# Autodesk Inventor assembly: GripE
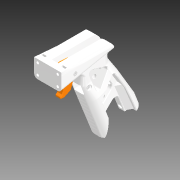
[picture p0: Inventor's stored thumbnail of the model, 180x180]
Saved by Autodesk Inventor 2020 (Build 240168000, 168)
## iProperties
Created: 2020-09-14
Part Number: GripE
Document SubType Name: Assembly
Designer: DDeGo
Author: DDeGo
Revision Number: PRODUCT_VERSION_IDPRODUCT_VERSION_DESCR
## Documents named in this file (5)
- C:\Users\DDeGo\Documents\Drew\Projects\Nerf Aim Assist\ESPER\GripE.iam
- C:\Users\DDeGo\Documents\Drew\Projects\Nerf Aim Assist\ESPER\GripE.ipt
- C:\Users\DDeGo\Documents\Drew\Projects\Nerf Aim Assist\ESPER\TriggerE.ipt
- C:\Users\DDeGo\Documents\Drew\Projects\Nerf Aim Assist\ESPER\90273A108.ipt
- C:\Users\DDeGo\Documents\Drew\Projects\Nerf Aim Assist\Cad\144 Tooth Herringbone Gear Base Mount.ipt
## Components (7 placed, 7 different names)
1. NAUO_ID9 — Flush:1, Flush:2, Mate:1, Mate:2
2. NAUO_ID29 — Mate:1, Mate:2
3. NAUO_ID69
4. NAUO_ID79
5. NAUO_ID99
6. NAUO_ID109
7. 144 Tooth Herringbone Gear Base Mount:1 — Flush:1, Flush:2
## Relationships (4: Flush 2, Mate 2)
- Flush:1: NAUO_ID9 ↔ 144 Tooth Herringbone Gear Base Mount:1
- Flush:2: NAUO_ID9 ↔ 144 Tooth Herringbone Gear Base Mount:1
- Mate:1: NAUO_ID9 ↔ NAUO_ID29
- Mate:2 (0.75 mm): NAUO_ID9 ↔ NAUO_ID29
